# Autodesk Inventor assembly: BBP
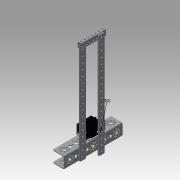
[picture p0: Inventor's stored thumbnail of the model, 180x180]
Saved by Autodesk Inventor 2016 (Build 200138000, 138)
## iProperties
Created: 2016-09-30
Part Number: BBP
Document SubType Name: Assembly
Designer: Delta
Author: Delta
## Documents named in this file (6)
- C:\Robotics\2016-17_CAD\BBP.iam
- C:\Robotics\CAD\2015-16\COTSParts\Tetrix\Tetrix channel 160mm.ipt
- C:\Robotics\CAD\2015-16\COTSParts\Tetrix\Tetrix flat bar 288mm.ipt
- C:\Robotics\CAD\2015-16\COTSParts\Tetrix\Tetrix bracket - single servo.ipt
- C:\Robotics\CAD\2015-16\COTSParts\Actobotics\585 parts\585382.ipt
- C:\Robotics\CAD\2015-16\COTSParts\Tetrix\Tetrix 180 Servo.ipt
## Components (6 placed, 5 different names)
1. Tetrix channel 160mm:2 — Insert:1, Insert:2, Insert:3
2. Tetrix flat bar 288mm:1 — Insert:1, Insert:4
3. Tetrix flat bar 288mm:2 — Insert:5
4. Tetrix bracket - single servo:1 — Insert:2, Insert:3, Insert:6
5. 585382:2 — Insert:4, Insert:5
6. Tetrix 180 Servo:1 — Insert:6
## Relationships (6: Insert 6)
- Insert:1: Tetrix channel 160mm:2 ↔ Tetrix flat bar 288mm:1
- Insert:2: Tetrix channel 160mm:2 ↔ Tetrix bracket - single servo:1
- Insert:3: Tetrix channel 160mm:2 ↔ Tetrix bracket - single servo:1
- Insert:4: Tetrix flat bar 288mm:1 ↔ 585382:2
- Insert:5: Tetrix flat bar 288mm:2 ↔ 585382:2
- Insert:6: Tetrix bracket - single servo:1 ↔ Tetrix 180 Servo:1
